# Autodesk Inventor assembly: 换向阀
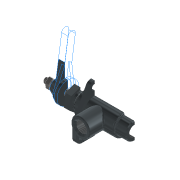
[picture p0: Inventor's stored thumbnail of the model, 180x180]
Saved by Autodesk Inventor 2022 (Build 260153000, 153)
## iProperties
Created: 2023-01-26
Part Number: 换向阀
Document SubType Name: Assembly
Designer: Lzy18
Author: Lzy18
## Documents named in this file (8)
- C:\Users\Lzy18\Desktop\换向阀\换向阀.iam
- C:\Users\Lzy18\Desktop\换向阀\1-阀体.ipt
- C:\Users\Lzy18\Desktop\换向阀\2-阀门.ipt
- C:\Users\Lzy18\Desktop\换向阀\3-锁紧螺母.ipt
- C:\Users\Lzy18\Desktop\换向阀\4-手柄.ipt
- C:\Users\Lzy18\Desktop\换向阀\6-螺母.ipt
- C:\Users\Lzy18\Documents\Inventor\Content Center Files\R2022\zh-CN\GB 93-87\垫圈 GB 93-87 8.ipt
- C:\Users\Lzy18\Desktop\巴雷特\零件2.ipt
## Components (7 placed, 7 different names)
1. 1-阀体:1 — 配合:11, 配合:13
2. 2-阀门:1 — 配合:8, 配合:9, 配合:10, 插入:2, 插入:3, 配合:11, 配合:12, 配合:14
3. 3-锁紧螺母:1 — 配合:12, 配合:13, 插入:4
4. 4-手柄:1 — 配合:8, 配合:9, 配合:10
5. 6-螺母:1 — 插入:3
6. 垫圈 GB/T 93-1987 M8:1 — 插入:2
7. 零件2:1 — 表面齐平:1, 插入:4, 配合:14
## Relationships (11: Mate 7, Insert 3, Flush 1)
- 配合:8 [Mate]: 2-阀门:1 ↔ 4-手柄:1
- 配合:9 [Mate]: 2-阀门:1 ↔ 4-手柄:1
- 配合:10 [Mate]: 2-阀门:1 ↔ 4-手柄:1
- 插入:2 [Insert]: 2-阀门:1 ↔ 垫圈 GB/T 93-1987 M8:1
- 插入:3 [Insert]: 2-阀门:1 ↔ 6-螺母:1
- 配合:11 [Mate]: 1-阀体:1 ↔ 2-阀门:1
- 配合:12 [Mate]: 2-阀门:1 ↔ 3-锁紧螺母:1
- 配合:13 [Mate] (7 mm): 1-阀体:1 ↔ 3-锁紧螺母:1
- 表面齐平:1 [Flush]: 零件2:1
- 插入:4 [Insert]: 3-锁紧螺母:1 ↔ 零件2:1
- 配合:14 [Mate]: 2-阀门:1 ↔ 零件2:1
